# Autodesk Inventor assembly: ZlozeniePrzegubu
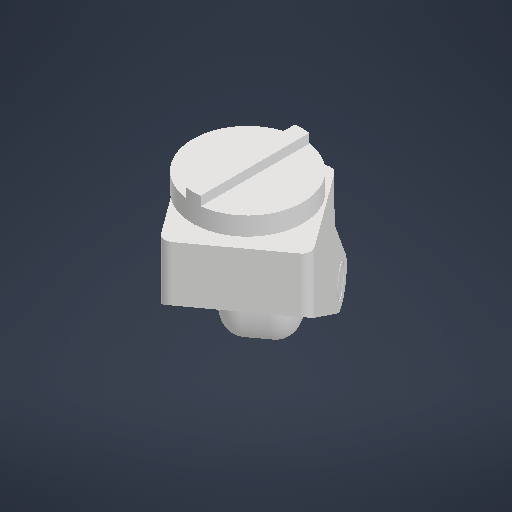
[picture p0: Inventor's stored thumbnail of the model, 512x512]
Saved by Autodesk Inventor 2026 (Build 300175000, 175)
## iProperties
Created: 2025-05-01
Part Number: ZlozeniePrzegubu
Document SubType Name: Assembly
Designer: isan
Author: isan
## Documents named in this file (6)
- E:\Conan II enhanced\ZlozeniePrzegubu.iam
- E:\Conan II enhanced\PrzegubGorny.ipt
- E:\Conan II enhanced\PrzegubDolny.ipt
- E:\Conan II enhanced\Kolek.ipt
- E:\Conan II enhanced\KolekNaKolo.ipt
- E:\Conan II enhanced\KoloPrzegubu.ipt
## Components (5 placed, 5 different names)
1. PrzegubGorny:1 — Mate:1, Mate:2
2. PrzegubDolny:1 — Mate:1, Mate:2, Mate:3, Mate:4, Mate:5, Flush:1, Mate:7
3. Kolek:1 — Mate:3, Mate:4
4. KolekNaKolo:1 — Mate:5, Flush:1, Mate:6
5. KoloPrzegubu:1 — Mate:6, Mate:7
## Relationships (8: Mate 7, Flush 1)
- Mate:1: PrzegubGorny:1 ↔ PrzegubDolny:1
- Mate:2 (0.1 mm): PrzegubGorny:1 ↔ PrzegubDolny:1
- Mate:3: PrzegubDolny:1 ↔ Kolek:1
- Mate:4: PrzegubDolny:1 ↔ Kolek:1
- Mate:5: PrzegubDolny:1 ↔ KolekNaKolo:1
- Flush:1: PrzegubDolny:1 ↔ KolekNaKolo:1
- Mate:6: KolekNaKolo:1 ↔ KoloPrzegubu:1
- Mate:7 (0.2 mm): PrzegubDolny:1 ↔ KoloPrzegubu:1
